# Autodesk Inventor assembly: Cabinet-FerriteCore
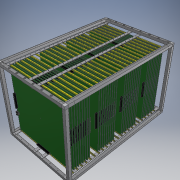
[picture p0: Inventor's stored thumbnail of the model, 180x180]
Saved by Autodesk Inventor 2018 (Build 220112000, 112)
## iProperties
Created: 2025-02-17
Part Number: Cabinet-FerriteCore
Material: Všeobecné
Document SubType Name: Assembly
Designer: Jozko Mrkvicka
Author: Jozko Mrkvicka
## Documents named in this file (9)
- D:\05_Projekty\Projects_Inventor\Haluska9000\Cabinet-FerriteCore.iam
- D:\05_Projekty\Projects_Inventor\Haluska9000\Profile-Connector.ipt
- D:\05_Projekty\Projects_Inventor\Haluska9000\Profile-Connector\Profile-Connector#15x15xCorner.ipt
- D:\05_Projekty\Projects_Inventor\Haluska9000\FerriteCoreMem-1KB.iam
- D:\05_Projekty\Projects_Inventor\Haluska9000\CardGuideArray-6-Inch.iam
- D:\05_Projekty\Projects_Inventor\Haluska9000\Profile-Square-Gray\Profile-Square#Cabinet-FerriteCore-Height.ipt
- D:\05_Projekty\Projects_Inventor\Haluska9000\Profile-Square-Gray\Profile-Square#Cabinet-FerriteCore-Width.ipt
- D:\05_Projekty\Projects_Inventor\Haluska9000\Profile-Square-Gray\Profile-Square#Cabinet-FerriteCore-Length.ipt
- D:\05_Projekty\Projects_Inventor\Haluska9000\Profile-Square-Gray.ipt
## Components (28 placed, 6 different names)
1. Profile-Square#Cabinet-FerriteCore-Height:14
2. Profile-Square#Cabinet-FerriteCore-Height:17
3. Profile-Square#Cabinet-FerriteCore-Height:20
4. Profile-Square#Cabinet-FerriteCore-Height:23
5. Profile-Square#Cabinet-FerriteCore-Width:15
6. Profile-Square#Cabinet-FerriteCore-Width:18
7. Profile-Square#Cabinet-FerriteCore-Width:21
8. Profile-Square#Cabinet-FerriteCore-Width:24
9. Profile-Square#Cabinet-FerriteCore-Length:13 — Proti sobě:324, Proti sobě:325, Stejný směr:38, Stejný směr:39, Proti sobě:326, Proti sobě:327
10. Profile-Square#Cabinet-FerriteCore-Length:16 — Stejný směr:35, Stejný směr:37, Proti sobě:320, Proti sobě:321, Proti sobě:322, Proti sobě:323
11. Profile-Square#Cabinet-FerriteCore-Length:19
12. Profile-Square#Cabinet-FerriteCore-Length:22
13. Profile-Connector#15x15xCorner:17
14. Profile-Connector#15x15xCorner:18
15. Profile-Connector#15x15xCorner:19
16. Profile-Connector#15x15xCorner:20
17. Profile-Connector#15x15xCorner:21
18. Profile-Connector#15x15xCorner:22
19. Profile-Connector#15x15xCorner:23
20. Profile-Connector#15x15xCorner:24
21. FerriteCoreMem-1KB:1 [sub-assembly] — Stejný směr:28, Stejný směr:31, Proti sobě:332
22. FerriteCoreMem-1KB:2 [sub-assembly] — Stejný směr:29, Stejný směr:30, Stejný směr:32, Stejný směr:33, Proti sobě:334
23. FerriteCoreMem-1KB:3 [sub-assembly] — Stejný směr:28, Stejný směr:29, Stejný směr:31, Stejný směr:32, Proti sobě:333
24. FerriteCoreMem-1KB:4 [sub-assembly] — Stejný směr:30, Stejný směr:33, Proti sobě:328, Proti sobě:329
25. CardGuideArray-6-Inch:1 [sub-assembly] — Stejný směr:35, Proti sobě:320, Proti sobě:322, Proti sobě:332, Proti sobě:333, Proti sobě:334
26. CardGuideArray-6-Inch:2 [sub-assembly] — Stejný směr:37, Proti sobě:321, Proti sobě:323, Proti sobě:328, Proti sobě:329
27. CardGuideArray-6-Inch:3 [sub-assembly] — Proti sobě:324, Stejný směr:38, Proti sobě:326
28. CardGuideArray-6-Inch:4 [sub-assembly] — Proti sobě:325, Stejný směr:39, Proti sobě:327
## Relationships (80: Mate 70, Flush 10)
- [Mate]: Profile-Square#Cabinet-FerriteCore-Length:13 ↔ Profile-Connector#15x15xCorner:17
- [Mate]: Profile-Square#Cabinet-FerriteCore-Length:13 ↔ Profile-Connector#15x15xCorner:17
- [Mate]: Profile-Square#Cabinet-FerriteCore-Length:13 ↔ Profile-Connector#15x15xCorner:17
- [Mate]: Profile-Square#Cabinet-FerriteCore-Height:14 ↔ Profile-Connector#15x15xCorner:17
- [Mate]: Profile-Square#Cabinet-FerriteCore-Height:14 ↔ Profile-Connector#15x15xCorner:17
- [Mate]: Profile-Square#Cabinet-FerriteCore-Height:14 ↔ Profile-Connector#15x15xCorner:17
- [Mate]: Profile-Square#Cabinet-FerriteCore-Width:15 ↔ Profile-Connector#15x15xCorner:17
- [Mate]: Profile-Square#Cabinet-FerriteCore-Width:15 ↔ Profile-Connector#15x15xCorner:17
- [Mate]: Profile-Square#Cabinet-FerriteCore-Width:15 ↔ Profile-Connector#15x15xCorner:17
- [Mate]: Profile-Square#Cabinet-FerriteCore-Length:13 ↔ Profile-Connector#15x15xCorner:18
- [Mate]: Profile-Square#Cabinet-FerriteCore-Length:13 ↔ Profile-Connector#15x15xCorner:18
- [Mate]: Profile-Square#Cabinet-FerriteCore-Length:13 ↔ Profile-Connector#15x15xCorner:18
- [Mate]: Profile-Square#Cabinet-FerriteCore-Length:16 ↔ Profile-Connector#15x15xCorner:19
- [Mate]: Profile-Square#Cabinet-FerriteCore-Length:16 ↔ Profile-Connector#15x15xCorner:19
- [Mate]: Profile-Square#Cabinet-FerriteCore-Length:16 ↔ Profile-Connector#15x15xCorner:19
- [Mate]: Profile-Square#Cabinet-FerriteCore-Height:17 ↔ Profile-Connector#15x15xCorner:19
- [Mate]: Profile-Square#Cabinet-FerriteCore-Height:17 ↔ Profile-Connector#15x15xCorner:19
- [Mate]: Profile-Square#Cabinet-FerriteCore-Height:17 ↔ Profile-Connector#15x15xCorner:19
- [Mate]: Profile-Square#Cabinet-FerriteCore-Width:18 ↔ Profile-Connector#15x15xCorner:19
- [Mate]: Profile-Square#Cabinet-FerriteCore-Width:18 ↔ Profile-Connector#15x15xCorner:19
- [Mate]: Profile-Square#Cabinet-FerriteCore-Width:18 ↔ Profile-Connector#15x15xCorner:19
- [Mate]: Profile-Square#Cabinet-FerriteCore-Length:16 ↔ Profile-Connector#15x15xCorner:20
- [Mate]: Profile-Square#Cabinet-FerriteCore-Length:16 ↔ Profile-Connector#15x15xCorner:20
- [Mate]: Profile-Square#Cabinet-FerriteCore-Length:16 ↔ Profile-Connector#15x15xCorner:20
- [Mate]: Profile-Square#Cabinet-FerriteCore-Height:17 ↔ Profile-Connector#15x15xCorner:18
- [Mate]: Profile-Square#Cabinet-FerriteCore-Height:17 ↔ Profile-Connector#15x15xCorner:18
- [Mate]: Profile-Square#Cabinet-FerriteCore-Height:17 ↔ Profile-Connector#15x15xCorner:18
- [Mate]: Profile-Square#Cabinet-FerriteCore-Length:19 ↔ Profile-Connector#15x15xCorner:21
- [Mate]: Profile-Square#Cabinet-FerriteCore-Length:19 ↔ Profile-Connector#15x15xCorner:21
- [Mate]: Profile-Square#Cabinet-FerriteCore-Length:19 ↔ Profile-Connector#15x15xCorner:21
- [Mate]: Profile-Square#Cabinet-FerriteCore-Height:20 ↔ Profile-Connector#15x15xCorner:21
- [Mate]: Profile-Square#Cabinet-FerriteCore-Height:20 ↔ Profile-Connector#15x15xCorner:21
- [Mate]: Profile-Square#Cabinet-FerriteCore-Height:20 ↔ Profile-Connector#15x15xCorner:21
- [Mate]: Profile-Square#Cabinet-FerriteCore-Width:21 ↔ Profile-Connector#15x15xCorner:21
- [Mate]: Profile-Square#Cabinet-FerriteCore-Width:21 ↔ Profile-Connector#15x15xCorner:21
- [Mate]: Profile-Square#Cabinet-FerriteCore-Width:21 ↔ Profile-Connector#15x15xCorner:21
- [Mate]: Profile-Square#Cabinet-FerriteCore-Length:19 ↔ Profile-Connector#15x15xCorner:22
- [Mate]: Profile-Square#Cabinet-FerriteCore-Length:19 ↔ Profile-Connector#15x15xCorner:22
- [Mate]: Profile-Square#Cabinet-FerriteCore-Length:19 ↔ Profile-Connector#15x15xCorner:22
- [Mate]: Profile-Square#Cabinet-FerriteCore-Length:22 ↔ Profile-Connector#15x15xCorner:23
- [Mate]: Profile-Square#Cabinet-FerriteCore-Length:22 ↔ Profile-Connector#15x15xCorner:23
- [Mate]: Profile-Square#Cabinet-FerriteCore-Length:22 ↔ Profile-Connector#15x15xCorner:23
- [Mate]: Profile-Square#Cabinet-FerriteCore-Height:23 ↔ Profile-Connector#15x15xCorner:23
- [Mate]: Profile-Square#Cabinet-FerriteCore-Height:23 ↔ Profile-Connector#15x15xCorner:23
- [Mate]: Profile-Square#Cabinet-FerriteCore-Height:23 ↔ Profile-Connector#15x15xCorner:23
- [Mate]: Profile-Square#Cabinet-FerriteCore-Width:24 ↔ Profile-Connector#15x15xCorner:23
- [Mate]: Profile-Square#Cabinet-FerriteCore-Width:24 ↔ Profile-Connector#15x15xCorner:23
- [Mate]: Profile-Square#Cabinet-FerriteCore-Width:24 ↔ Profile-Connector#15x15xCorner:23
- [Mate]: Profile-Square#Cabinet-FerriteCore-Length:22 ↔ Profile-Connector#15x15xCorner:24
- [Mate]: Profile-Square#Cabinet-FerriteCore-Length:22 ↔ Profile-Connector#15x15xCorner:24
- [Mate]: Profile-Square#Cabinet-FerriteCore-Length:22 ↔ Profile-Connector#15x15xCorner:24
- [Mate]: Profile-Square#Cabinet-FerriteCore-Height:23 ↔ Profile-Connector#15x15xCorner:22
- [Mate]: Profile-Square#Cabinet-FerriteCore-Height:23 ↔ Profile-Connector#15x15xCorner:22
- [Mate]: Profile-Square#Cabinet-FerriteCore-Height:23 ↔ Profile-Connector#15x15xCorner:22
- [Mate]: Profile-Square#Cabinet-FerriteCore-Width:21 ↔ Profile-Connector#15x15xCorner:18
- [Mate]: Profile-Square#Cabinet-FerriteCore-Width:21 ↔ Profile-Connector#15x15xCorner:18
- [Mate]: Profile-Square#Cabinet-FerriteCore-Width:21 ↔ Profile-Connector#15x15xCorner:18
- Stejný směr:28 [Flush]: FerriteCoreMem-1KB:1 ↔ FerriteCoreMem-1KB:3
- Stejný směr:29 [Flush]: FerriteCoreMem-1KB:2 ↔ FerriteCoreMem-1KB:3
- Stejný směr:30 [Flush]: FerriteCoreMem-1KB:2 ↔ FerriteCoreMem-1KB:4
- Stejný směr:31 [Flush]: FerriteCoreMem-1KB:1 ↔ FerriteCoreMem-1KB:3
- Stejný směr:32 [Flush]: FerriteCoreMem-1KB:2 ↔ FerriteCoreMem-1KB:3
- Stejný směr:33 [Flush]: FerriteCoreMem-1KB:2 ↔ FerriteCoreMem-1KB:4
- Stejný směr:35 [Flush]: Profile-Square#Cabinet-FerriteCore-Length:16 ↔ CardGuideArray-6-Inch:1
- Stejný směr:37 [Flush]: Profile-Square#Cabinet-FerriteCore-Length:16 ↔ CardGuideArray-6-Inch:2
- Proti sobě:320 [Mate]: Profile-Square#Cabinet-FerriteCore-Length:16 ↔ CardGuideArray-6-Inch:1
- Proti sobě:321 [Mate]: Profile-Square#Cabinet-FerriteCore-Length:16 ↔ CardGuideArray-6-Inch:2
- Proti sobě:322 [Mate]: Profile-Square#Cabinet-FerriteCore-Length:16 ↔ CardGuideArray-6-Inch:1
- Proti sobě:323 [Mate]: Profile-Square#Cabinet-FerriteCore-Length:16 ↔ CardGuideArray-6-Inch:2
- Proti sobě:324 [Mate]: Profile-Square#Cabinet-FerriteCore-Length:13 ↔ CardGuideArray-6-Inch:3
- Proti sobě:325 [Mate]: Profile-Square#Cabinet-FerriteCore-Length:13 ↔ CardGuideArray-6-Inch:4
- Stejný směr:38 [Flush]: Profile-Square#Cabinet-FerriteCore-Length:13 ↔ CardGuideArray-6-Inch:3
- Stejný směr:39 [Flush]: Profile-Square#Cabinet-FerriteCore-Length:13 ↔ CardGuideArray-6-Inch:4
- Proti sobě:326 [Mate]: Profile-Square#Cabinet-FerriteCore-Length:13 ↔ CardGuideArray-6-Inch:3
- Proti sobě:327 [Mate]: Profile-Square#Cabinet-FerriteCore-Length:13 ↔ CardGuideArray-6-Inch:4
- Proti sobě:328 [Mate]: FerriteCoreMem-1KB:4 ↔ CardGuideArray-6-Inch:2
- Proti sobě:329 [Mate]: FerriteCoreMem-1KB:4 ↔ CardGuideArray-6-Inch:2
- Proti sobě:332 [Mate]: FerriteCoreMem-1KB:1 ↔ CardGuideArray-6-Inch:1
- Proti sobě:333 [Mate]: FerriteCoreMem-1KB:3 ↔ CardGuideArray-6-Inch:1
- Proti sobě:334 [Mate]: FerriteCoreMem-1KB:2 ↔ CardGuideArray-6-Inch:1
## Named parameters: d485_d297 = 0 mm, d486_d298 = 0 mm, d487_d299 = 0 mm, d490_d245 = 0 mm, d491_d246 = 0 mm, d492_d247 = 0 mm, d493_d248 = 0 mm, d494_d249 = 0 mm, d495_d250 = 0 mm, d496_d251 = 0 mm, d497_d252 = 0 mm, d498_d253 = 0 mm, d499_d254 = 0 mm, d500_d255_d243 = 0 mm, d501_d256_d244 = 0 mm, d502_d257_d245 = 0 mm, d503_d258_d246 = 0 mm, d504_d259_d247 = 0 mm, d505_d260_d248 = 0 mm, d506_d261_d249 = 0 mm, d507_d262_d250 = 0 mm, d508_d263_d251 = 0 mm, d509_d264_d252 = 0 mm, d510_d265_d253 = 0 mm, d511_d266_d254 = 0 mm, d512_d267 = 0 mm, d513_d268 = 0 mm, d514_d269 = 0 mm, d515_d270_d260_d248 = 0 mm, d516_d271_d261_d249 = 0 mm, d517_d272_d262_d250 = 0 mm, d518_d273_d263_d251 = 0 mm, d519_d274_d264_d252 = 0 mm, d520_d275_d265_d253 = 0 mm, d521_d276_d266_d254 = 0 mm, d522_d277_d267 = 0 mm, d523_d278_d268 = 0 mm, d524_d279_d269 = 0 mm, d525_d280_d243 = 0 mm, d526_d281_d244 = 0 mm, d527_d282_d245 = 0 mm, d528_d283_d246 = 0 mm, d529_d284_d247 = 0 mm, d530_d285_d248 = 0 mm, d531_d286_d249 = 0 mm, d532_d287_d250 = 0 mm, d533_d288_d251 = 0 mm, d534_d289_d252 = 0 mm, d535_d290_d253 = 0 mm, d536_d291_d254 = 0 mm, d537_d292_d255_d243 = 0 mm, d538_d293_d256_d244 = 0 mm, d539_d294_d257_d245 = 0 mm, d540_d295_d258_d246 = 0 mm, d541_d296_d259_d247 = 0 mm, d542_d243 = 0 mm, d543_d244 = 0 mm
